# Autodesk Inventor assembly: head_link
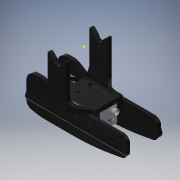
[picture p0: Inventor's stored thumbnail of the model, 180x180]
Saved by Autodesk Inventor 2018 (Build 220112000, 112)
## iProperties
Created: 2018-12-01
Part Number: head_link
Document SubType Name: Assembly
Designer: jaspe
Author: jaspe
## Documents named in this file (5)
- C:\Users\bitbots\Desktop\bitbots_hardware\wolfgang\assembly\head\head_link.iam
- C:\Users\bitbots\Desktop\bitbots_hardware\wolfgang\assembly\head\camera_lower_baseler_wolfgang_v2.1.ipt
- C:\Users\bitbots\Desktop\bitbots_hardware\wolfgang\assembly\head\camera_side_basler_wolfgang_v2.2.ipt
- C:\Users\bitbots\Desktop\bitbots_hardware\wolfgang\assembly\head\camera_side_basler_wolfgang_v2.2_MIR.ipt
- C:\Users\bitbots\Desktop\bitbots_hardware\camera\camera_and_lens.iam
## Components (4 placed, 4 different names)
1. camera_lower_baseler_wolfgang_v2.1:1 — Mate:1, Mate:2, Angle:1, Mate:3, Mate:4, Mate:5, Mate:6, Mate:7, Mate:8, Mate:9, Mate:10, Mate:11
2. camera_side_basler_wolfgang_v2.2:1 — Mate:6, Mate:7, Mate:8
3. camera_side_basler_wolfgang_v2.2_MIR:1 — Mate:3, Mate:4, Mate:5
4. camera_and_lens:1 [sub-assembly] — Mate:9, Mate:10, Mate:11
## Relationships (12: Mate 11, Angle 1)
- Mate:1: camera_lower_baseler_wolfgang_v2.1:1
- Mate:2: camera_lower_baseler_wolfgang_v2.1:1
- Angle:1 (0 deg): camera_lower_baseler_wolfgang_v2.1:1
- Mate:3: camera_lower_baseler_wolfgang_v2.1:1 ↔ camera_side_basler_wolfgang_v2.2_MIR:1
- Mate:4: camera_lower_baseler_wolfgang_v2.1:1 ↔ camera_side_basler_wolfgang_v2.2_MIR:1
- Mate:5: camera_lower_baseler_wolfgang_v2.1:1 ↔ camera_side_basler_wolfgang_v2.2_MIR:1
- Mate:6: camera_lower_baseler_wolfgang_v2.1:1 ↔ camera_side_basler_wolfgang_v2.2:1
- Mate:7: camera_lower_baseler_wolfgang_v2.1:1 ↔ camera_side_basler_wolfgang_v2.2:1
- Mate:8: camera_lower_baseler_wolfgang_v2.1:1 ↔ camera_side_basler_wolfgang_v2.2:1
- Mate:9: camera_lower_baseler_wolfgang_v2.1:1 ↔ camera_and_lens:1
- Mate:10: camera_lower_baseler_wolfgang_v2.1:1 ↔ camera_and_lens:1
- Mate:11: camera_lower_baseler_wolfgang_v2.1:1 ↔ camera_and_lens:1
